# Autodesk Inventor assembly: Linearfuehrung Bosch Rexroth R0442
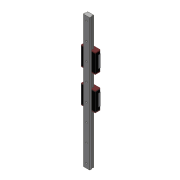
[picture p0: Inventor's stored thumbnail of the model, 180x180]
Saved by Autodesk Inventor 2016 (Build 200138000, 138)
## iProperties
Created: 2015-07-20
Part Number: Linearfuehrung Bosch Rexroth R0442
Document SubType Name: Assembly
## Documents named in this file (3)
- E:\GitHub\CNC-Router_Z-Axis\Linearfuehrung Bosch Rexroth R0442.iam
- E:\GitHub\CNC-Router_Z-Axis\R044550331_300.ipt
- E:\GitHub\CNC-Router_Z-Axis\R0442-15.ipt
## Components (3 placed, 2 different names)
1. R044550331_300:1 — Mate:1, Mate:2, Mate:3, Mate:4
2. R0442-15:1 — Mate:1, Mate:2
3. R0442-15:2 — Mate:3, Mate:4
## Relationships (4: Mate 4)
- Mate:1: R044550331_300:1 ↔ R0442-15:1
- Mate:2: R044550331_300:1 ↔ R0442-15:1
- Mate:3: R044550331_300:1 ↔ R0442-15:2
- Mate:4: R044550331_300:1 ↔ R0442-15:2
